# Autodesk Inventor assembly: artschallenge2022c
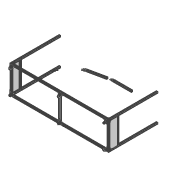
[picture p0: Inventor's stored thumbnail of the model, 180x180]
Saved by Autodesk Inventor 2020 (Build 240168000, 168)
## iProperties
Created: 2021-11-28
Part Number: artschallenge2022c
Description: CAx-IF Rec.Pracs.---Model Styling and Organization---1.2---2011-12-15
Document SubType Name: Assembly
Designer: ken113
Sending System: 3D_Kernel_IO2017 Sp2 by CT CoreTechnologie
Preprocessor: STEP Interface 2017 Sp2 by CT CoreTechnologie
Title: artschallenge2022c.stp
## Documents named in this file (32)
- D:\Document\Github\Eto_Project\Hardware\Parts\MISUMI_FRAMES\artschallenge2022c.iam
- D:\Document\Github\Eto_Project\Hardware\Parts\MISUMI_FRAMES\NEFSB8-5050-2800.ipt
- D:\Document\Github\Eto_Project\Hardware\Parts\MISUMI_FRAMES\HFSB8-5050-706.ipt
- D:\Document\Github\Eto_Project\Hardware\Parts\MISUMI_FRAMES\HFSB8-5050-1350.ipt
- D:\Document\Github\Eto_Project\Hardware\Parts\MISUMI_FRAMES\HBKTSB8-SET(1).iam
- D:\Document\Github\Eto_Project\Hardware\Parts\MISUMI_FRAMES\HBKTSB8-SET(2).iam
- D:\Document\Github\Eto_Project\Hardware\Parts\MISUMI_FRAMES\HBKTSB8-SET(3).iam
- D:\Document\Github\Eto_Project\Hardware\Parts\MISUMI_FRAMES\HBKTSB8-SET(4).iam
- D:\Document\Github\Eto_Project\Hardware\Parts\MISUMI_FRAMES\HBKTSB8-SET(5).iam
- D:\Document\Github\Eto_Project\Hardware\Parts\MISUMI_FRAMES\HBKTSB8-SET(6).iam
- D:\Document\Github\Eto_Project\Hardware\Parts\MISUMI_FRAMES\HBKTSB8-SET(7).iam
- D:\Document\Github\Eto_Project\Hardware\Parts\MISUMI_FRAMES\HBKTSB8-SET(8).iam
- D:\Document\Github\Eto_Project\Hardware\Parts\MISUMI_FRAMES\HCHJF65-N.iam
- D:\Document\Github\Eto_Project\Hardware\Parts\MISUMI_FRAMES\HBKTSB8-SET(9).iam
- D:\Document\Github\Eto_Project\Hardware\Parts\MISUMI_FRAMES\HBKTSB8-SET(10).iam
- D:\Document\Github\Eto_Project\Hardware\Parts\MISUMI_FRAMES\HBKTSB8-SET(11).iam
- D:\Document\Github\Eto_Project\Hardware\Parts\MISUMI_FRAMES\HBKTSB8-SET(12).iam
- D:\Document\Github\Eto_Project\Hardware\Parts\MISUMI_FRAMES\HBKTSB8-SET(13).iam
- D:\Document\Github\Eto_Project\Hardware\Parts\MISUMI_FRAMES\HBKTSB8-SET(14).iam
- D:\Document\Github\Eto_Project\Hardware\Parts\MISUMI_FRAMES\HBKTSB8-SET(15).iam
- D:\Document\Github\Eto_Project\Hardware\Parts\MISUMI_FRAMES\HBKTSB8-SET(16).iam
- D:\Document\Github\Eto_Project\Hardware\Parts\MISUMI_FRAMES\HBKTSB8-SET(17).iam
- D:\Document\Github\Eto_Project\Hardware\Parts\MISUMI_FRAMES\HBKTSB8-SET(18).iam
- D:\Document\Github\Eto_Project\Hardware\Parts\MISUMI_FRAMES\HBKTSB8-SET(19).iam
- D:\Document\Github\Eto_Project\Hardware\Parts\MISUMI_FRAMES\HBKTSB8-SET(20).iam
- D:\Document\Github\Eto_Project\Hardware\Parts\MISUMI_FRAMES\L-PCTA(Non-Standard)(1).ipt
- D:\Document\Github\Eto_Project\Hardware\Parts\MISUMI_FRAMES\L-PCTA(Non-Standard)(2).ipt
- D:\Document\Github\Eto_Project\Hardware\Parts\MISUMI_FRAMES\HNTT8-8.ipt
- D:\Document\Github\Eto_Project\Hardware\Parts\MISUMI_FRAMES\CBM8-12.ipt
- D:\Document\Github\Eto_Project\Hardware\Parts\MISUMI_FRAMES\HCBM5-8.ipt
- D:\Document\Github\Eto_Project\Hardware\Parts\MISUMI\HBLTBBN45-SET_Autodesk_Inventor_2020_20211206\AIS2020\HBLTBBN45.iam
- D:\Document\Github\Eto_Project\Hardware\Parts\MISUMI\HFS8-5050-500-LSV-RSV_Autodesk_Inventor_2020_20211206\HFS8-5050-500-LSV-RSV.ipt
## Components (100 placed, 31 different names)
1. NEFSB8-5050-2800
2. NEFSB8-5050-2800:1 — フラッシュ:11, メイト:5, フラッシュ:22
3. HFSB8-5050-706 — メイト:9
4. HFSB8-5050-706:1
5. HFSB8-5050-1350
6. HBKTSB8-SET(1) [sub-assembly]
7. HFSB8-5050-1350:1 — フラッシュ:17, メイト:11
8. HBKTSB8-SET(2) [sub-assembly]
9. HFSB8-5050-1350:2 — メイト:2, フラッシュ:6, フラッシュ:7, フラッシュ:16
10. HBKTSB8-SET(3) [sub-assembly]
11. HFSB8-5050-1350:3 — メイト:10
12. HBKTSB8-SET(4) [sub-assembly]
13. HFSB8-5050-706:2 — フラッシュ:12
14. HBKTSB8-SET(5) [sub-assembly]
15. HBKTSB8-SET(6) [sub-assembly]
16. HBKTSB8-SET(7) [sub-assembly]
17. HBKTSB8-SET(8) [sub-assembly]
18. HCHJF65-N [sub-assembly]
19. HCHJF65-N:1 [sub-assembly]
20. HFSB8-5050-706:3 — フラッシュ:16, メイト:9, メイト:10, フラッシュ:18
21. HBKTSB8-SET(9) [sub-assembly]
22. HBKTSB8-SET(10) [sub-assembly]
23. HFSB8-5050-706:4 — フラッシュ:17, メイト:11, フラッシュ:18
24. HBKTSB8-SET(11) [sub-assembly]
25. HBKTSB8-SET(12) [sub-assembly]
26. HBKTSB8-SET(13) [sub-assembly]
27. HBKTSB8-SET(14) [sub-assembly]
28. HBKTSB8-SET(15) [sub-assembly]
29. HBKTSB8-SET(16) [sub-assembly]
30. HBKTSB8-SET(17) [sub-assembly]
31. HBKTSB8-SET(18) [sub-assembly]
32. HBKTSB8-SET(19) [sub-assembly]
33. HBKTSB8-SET(20) [sub-assembly]
34. HCHJF65-N:2 [sub-assembly]
35. HCHJF65-N:3 [sub-assembly]
36. HCHJF65-N:4 [sub-assembly]
37. HCHJF65-N:5 [sub-assembly]
38. L-PCTA(Non-Standard)(1)
39. L-PCTA(Non-Standard)(2)
40. HNTT8-8
41. CBM8-12
42. HNTT8-8:1
43. CBM8-12:1
44. HNTT8-8:2
45. CBM8-12:2
46. HNTT8-8:3
47. CBM8-12:3
48. HNTT8-8:4
49. CBM8-12:4
50. HNTT8-8:5
51. CBM8-12:5
52. HNTT8-8:6
53. CBM8-12:6
54. HNTT8-8:7
55. CBM8-12:7
56. HNTT8-8:8
57. CBM8-12:8
58. HNTT8-8:9
59. CBM8-12:9
60. HNTT8-8:10
61. CBM8-12:10
62. HNTT8-8:11
63. CBM8-12:11
64. HNTT8-8:12
65. CBM8-12:12
66. HNTT8-8:13
67. CBM8-12:13
68. HNTT8-8:14
69. CBM8-12:14
70. HNTT8-8:15
71. CBM8-12:15
72. HNTT8-8:16
73. CBM8-12:16
74. HNTT8-8:17
75. CBM8-12:17
76. HNTT8-8:18
77. CBM8-12:18
78. HNTT8-8:19
79. CBM8-12:19
80. HNTT8-8:20
81. CBM8-12:20
82. HNTT8-8:21
83. CBM8-12:21
84. HNTT8-8:22
85. CBM8-12:22
86. HNTT8-8:23
87. CBM8-12:23
88. HCBM5-8
89. HCBM5-8:1
90. HCBM5-8:2
91. HCBM5-8:3
92. HCBM5-8:4
93. HCBM5-8:5
94. HCBM5-8:6
95. HCBM5-8:7
96. HBLTBBN45:2 [sub-assembly] — メイト:2, フラッシュ:6, フラッシュ:7, フラッシュ:8, フラッシュ:9, メイト:15
97. HBLTBBN45:3 [sub-assembly] — フラッシュ:8, フラッシュ:9, フラッシュ:15, メイト:12, フラッシュ:21, メイト:14, メイト:15
98. HFS8-5050-500-LSV-RSV:2 — フラッシュ:11, フラッシュ:12, メイト:5, フラッシュ:13, フラッシュ:14, フラッシュ:20
99. HBLTBBN45:4 [sub-assembly] — フラッシュ:13, フラッシュ:14, フラッシュ:15, メイト:14, フラッシュ:23
100. HFS8-5050-500-LSV-RSV:4 — メイト:12, フラッシュ:20, フラッシュ:21
## Relationships (24: Flush 16, Mate 8)
- メイト:2 [Mate] (-200 mm): HFSB8-5050-1350:2 ↔ HBLTBBN45:2
- フラッシュ:6 [Flush] (2.5 mm): HFSB8-5050-1350:2 ↔ HBLTBBN45:2
- フラッシュ:7 [Flush] (-2.5 mm): HFSB8-5050-1350:2 ↔ HBLTBBN45:2
- フラッシュ:8 [Flush]: HBLTBBN45:2 ↔ HBLTBBN45:3
- フラッシュ:9 [Flush]: HBLTBBN45:2 ↔ HBLTBBN45:3
- フラッシュ:11 [Flush]: NEFSB8-5050-2800:1 ↔ HFS8-5050-500-LSV-RSV:2
- フラッシュ:12 [Flush] (-225 mm): HFSB8-5050-706:2 ↔ HFS8-5050-500-LSV-RSV:2
- メイト:5 [Mate] (1740 mm): NEFSB8-5050-2800:1 ↔ HFS8-5050-500-LSV-RSV:2
- フラッシュ:13 [Flush] (2.5 mm): HFS8-5050-500-LSV-RSV:2 ↔ HBLTBBN45:4
- フラッシュ:14 [Flush] (-2.5 mm): HFS8-5050-500-LSV-RSV:2 ↔ HBLTBBN45:4
- フラッシュ:15 [Flush]: HBLTBBN45:3 ↔ HBLTBBN45:4
- フラッシュ:16 [Flush]: HFSB8-5050-1350:2 ↔ HFSB8-5050-706:3
- メイト:9 [Mate] (200 mm): HFSB8-5050-706 ↔ HFSB8-5050-706:3
- メイト:10 [Mate]: HFSB8-5050-1350:3 ↔ HFSB8-5050-706:3
- フラッシュ:17 [Flush]: HFSB8-5050-1350:1 ↔ HFSB8-5050-706:4
- メイト:11 [Mate]: HFSB8-5050-1350:1 ↔ HFSB8-5050-706:4
- フラッシュ:18 [Flush]: HFSB8-5050-706:3 ↔ HFSB8-5050-706:4
- メイト:12 [Mate]: HBLTBBN45:3 ↔ HFS8-5050-500-LSV-RSV:4
- フラッシュ:20 [Flush]: HFS8-5050-500-LSV-RSV:2 ↔ HFS8-5050-500-LSV-RSV:4
- フラッシュ:21 [Flush] (2.5 mm): HBLTBBN45:3 ↔ HFS8-5050-500-LSV-RSV:4
- メイト:14 [Mate] (600 mm): HBLTBBN45:3 ↔ HBLTBBN45:4
- メイト:15 [Mate] (550 mm): HBLTBBN45:2 ↔ HBLTBBN45:3
- フラッシュ:22 [Flush] (-1400 mm): NEFSB8-5050-2800:1
- フラッシュ:23 [Flush] (250 mm): HBLTBBN45:4
